# Autodesk Inventor assembly: disassembled
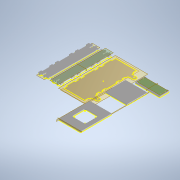
[picture p0: Inventor's stored thumbnail of the model, 180x180]
Saved by Autodesk Inventor 2020 (Build 240168000, 168)
## iProperties
Created: 2020-01-09
Part Number: disassembled
Document SubType Name: Assembly
Designer: erwin
Author: erwin
## Documents named in this file (8)
- D:\GitHub\ElCheapoAIS-nmea\case\Wooden Multicase\disassembled.iam
- D:\GitHub\ElCheapoAIS-nmea\case\Wooden Multicase\side_top.ipt
- D:\GitHub\ElCheapoAIS-nmea\case\Wooden Multicase\side_side.ipt
- D:\GitHub\ElCheapoAIS-nmea\case\Wooden Multicase\side_bottom.ipt
- D:\GitHub\ElCheapoAIS-nmea\case\Wooden Multicase\cover_wires.ipt
- D:\GitHub\ElCheapoAIS-nmea\case\Wooden Multicase\cover_components.ipt
- D:\GitHub\ElCheapoAIS-nmea\case\Wooden Multicase\prototype\cover.ipt
- D:\GitHub\ElCheapoAIS-nmea\case\Wooden Multicase\drawings_easel.ipt
## Components (8 placed, 7 different names)
1. side_top:1 — Mate:4
2. side_side:1 — Mate:6
3. side_side:2 — Mate:5
4. side_bottom:1 — Mate:3, Mate:4
5. cover_wires:1 — Mate:1, Mate:3
6. cover_components:1 — Mate:2
7. cover:1 — Mate:1, Mate:2, Mate:5, Mate:6, Flush:1, Flush:2, Flush:3
8. drawings_easel:1 — Flush:1, Flush:2, Flush:3
## Relationships (9: Mate 6, Flush 3)
- Mate:1: cover_wires:1 ↔ cover:1
- Mate:2: cover_components:1 ↔ cover:1
- Mate:3: side_bottom:1 ↔ cover_wires:1
- Mate:4: side_top:1 ↔ side_bottom:1
- Mate:5: side_side:2 ↔ cover:1
- Mate:6: side_side:1 ↔ cover:1
- Flush:1: cover:1 ↔ drawings_easel:1
- Flush:2: cover:1 ↔ drawings_easel:1
- Flush:3: cover:1 ↔ drawings_easel:1
